# Autodesk Inventor assembly: EnsamblajeCanSat_3
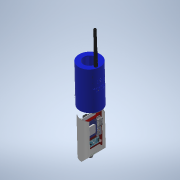
[picture p0: Inventor's stored thumbnail of the model, 180x180]
Saved by Autodesk Inventor 2021.3 (Build 253353010, 353A)
## iProperties
Created: 2021-08-20
Part Number: EnsamblajeCanSat_3
Document SubType Name: Assembly
Designer: pili2
Author: pili2
## Documents named in this file (13)
- C:\Users\pili2\OneDrive\Desktop\IRVI\EnsamblajeCanSat_3.iam
- C:\Users\pili2\OneDrive\Desktop\IRVI\cansat_estructura3.ipt
- C:\Users\pili2\OneDrive\Desktop\IRVI\tapa_estructura_3.ipt
- C:\Users\pili2\OneDrive\Desktop\IRVI\Bateria LiPo 3.7V 1000mA 503450 v23.ipt
- C:\Users\pili2\OneDrive\Desktop\IRVI\ARDUINO NANO - A000005.ipt
- C:\Users\pili2\OneDrive\Desktop\IRVI\MRO GPS.ipt
- C:\Users\pili2\OneDrive\Desktop\IRVI\IMU.ipt
- C:\Users\pili2\OneDrive\Desktop\IRVI\Antena 3 dBi 5.8 GHz v3.ipt
- C:\Users\pili2\OneDrive\Desktop\IRVI\OrangePi_Zero_LTS.ipt
- C:\Users\pili2\OneDrive\Desktop\IRVI\DC-DC XL6009E1.ipt
- C:\Users\pili2\OneDrive\Desktop\IRVI\Cam V2.1 v1.ipt
- C:\Users\pili2\OneDrive\Desktop\IRVI\DHT11 Temperatursensor.ipt
- C:\Users\pili2\OneDrive\Desktop\IRVI\Tapa baterías.ipt
## Components (15 placed, 12 different names)
1. cansat_estructura3:1 — Mate:3, Mate:4, Mate:5, Mate:9, Mate:10, Mate:11, Mate:12, Mate:13, Mate:14, Mate:21, Mate:22, Mate:29, Mate:30, Mate:31, Mate:32, Mate:33, Mate:34, Mate:37, Mate:39, Mate:42
2. tapa_estructura_3:1 — Mate:21, Mate:22, Mate:27, Mate:28, Mate:43, Mate:44, Mate:45, Mate:46, Mate:47, Mate:48, Mate:49, Mate:50, Mate:51, Mate:52, Mate:53, Mate:55, Mate:56, Mate:57, Mate:58
3. Bateria LiPo 3.7V 1000mA 503450 v23:1 — Mate:43, Mate:45, Mate:47
4. ARDUINO NANO - A000005:1 — Mate:3, Mate:4, Mate:5
5. MRO GPS:1 — Mate:9, Mate:10, Mate:11, Mate:40
6. IMU:1 — Mate:12, Mate:13, Mate:14, Mate:41
7. Antena 3 dBi 5.8 GHz v3:1 — Mate:27, Mate:28
8. OrangePi_Zero_LTS:1 — Mate:29, Mate:30, Mate:31
9. DC-DC XL6009E1:1 — Mate:32, Mate:33, Mate:34
10. Cam V2.1 v1:1 — Mate:37, Mate:42
11. DHT11 Temperatursensor:1 — Mate:39, Mate:40, Mate:41
12. Bateria LiPo 3.7V 1000mA 503450 v23:2 — Mate:44, Mate:46, Mate:48
13. Bateria LiPo 3.7V 1000mA 503450 v23:3 — Mate:49, Mate:50, Mate:51
14. Tapa baterías:1 — Mate:52, Mate:53, Mate:58
15. Tapa baterías:2 — Mate:55, Mate:56, Mate:57
## Relationships (39: Mate 39)
- Mate:3 (2 mm): cansat_estructura3:1 ↔ ARDUINO NANO - A000005:1
- Mate:4 (15 mm): cansat_estructura3:1 ↔ ARDUINO NANO - A000005:1
- Mate:5 (-25 mm): cansat_estructura3:1 ↔ ARDUINO NANO - A000005:1
- Mate:9 (2 mm): cansat_estructura3:1 ↔ MRO GPS:1
- Mate:10 (41 mm): cansat_estructura3:1 ↔ MRO GPS:1
- Mate:11 (-28 mm): cansat_estructura3:1 ↔ MRO GPS:1
- Mate:12: cansat_estructura3:1 ↔ IMU:1
- Mate:13 (33 mm): cansat_estructura3:1 ↔ IMU:1
- Mate:14 (-28 mm): cansat_estructura3:1 ↔ IMU:1
- Mate:21 (130 mm): cansat_estructura3:1 ↔ tapa_estructura_3:1
- Mate:22: cansat_estructura3:1 ↔ tapa_estructura_3:1
- Mate:27: tapa_estructura_3:1 ↔ Antena 3 dBi 5.8 GHz v3:1
- Mate:28 (-27 mm): tapa_estructura_3:1 ↔ Antena 3 dBi 5.8 GHz v3:1
- Mate:29: cansat_estructura3:1 ↔ OrangePi_Zero_LTS:1
- Mate:30 (25 mm): cansat_estructura3:1 ↔ OrangePi_Zero_LTS:1
- Mate:31 (-18 mm): cansat_estructura3:1 ↔ OrangePi_Zero_LTS:1
- Mate:32: cansat_estructura3:1 ↔ DC-DC XL6009E1:1
- Mate:33 (77 mm): cansat_estructura3:1 ↔ DC-DC XL6009E1:1
- Mate:34 (-20 mm): cansat_estructura3:1 ↔ DC-DC XL6009E1:1
- Mate:37: cansat_estructura3:1 ↔ Cam V2.1 v1:1
- Mate:39: cansat_estructura3:1 ↔ DHT11 Temperatursensor:1
- Mate:40: MRO GPS:1 ↔ DHT11 Temperatursensor:1
- Mate:41 (4 mm): IMU:1 ↔ DHT11 Temperatursensor:1
- Mate:42 (-0.2 mm): cansat_estructura3:1 ↔ Cam V2.1 v1:1
- Mate:43: tapa_estructura_3:1 ↔ Bateria LiPo 3.7V 1000mA 503450 v23:1
- Mate:44 (3 mm): tapa_estructura_3:1 ↔ Bateria LiPo 3.7V 1000mA 503450 v23:2
- Mate:45 (3 mm): tapa_estructura_3:1 ↔ Bateria LiPo 3.7V 1000mA 503450 v23:1
- Mate:46 (70 mm): tapa_estructura_3:1 ↔ Bateria LiPo 3.7V 1000mA 503450 v23:2
- Mate:47 (-10 mm): tapa_estructura_3:1 ↔ Bateria LiPo 3.7V 1000mA 503450 v23:1
- Mate:48 (-10 mm): tapa_estructura_3:1 ↔ Bateria LiPo 3.7V 1000mA 503450 v23:2
- Mate:49 (3 mm): tapa_estructura_3:1 ↔ Bateria LiPo 3.7V 1000mA 503450 v23:3
- Mate:50 (60 mm): tapa_estructura_3:1 ↔ Bateria LiPo 3.7V 1000mA 503450 v23:3
- Mate:51 (-10 mm): tapa_estructura_3:1 ↔ Bateria LiPo 3.7V 1000mA 503450 v23:3
- Mate:52: tapa_estructura_3:1 ↔ Tapa baterías:1
- Mate:53: tapa_estructura_3:1 ↔ Tapa baterías:1
- Mate:55: tapa_estructura_3:1 ↔ Tapa baterías:2
- Mate:56: tapa_estructura_3:1 ↔ Tapa baterías:2
- Mate:57: tapa_estructura_3:1 ↔ Tapa baterías:2
- Mate:58: tapa_estructura_3:1 ↔ Tapa baterías:1
